# Autodesk Inventor assembly: horas_40
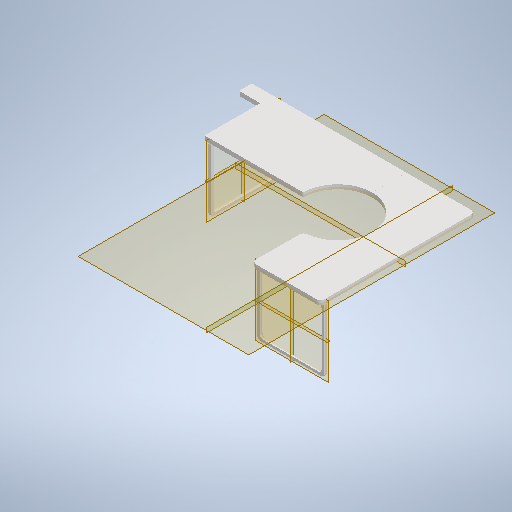
[picture p0: Inventor's stored thumbnail of the model, 512x512]
Saved by Autodesk Inventor 2025.2 (Build 292293000, 293)
## iProperties
Created: 2025-04-07
Part Number: horas_40
Document SubType Name: Assembly
Designer: kenay
Author: kenay
## Documents named in this file (4)
- C:\Users\kenay\Documents\Aula 40horas\horas_40.iam
- C:\Users\kenay\Documents\Aula 40horas\Lado Esquerdo Mesa.ipt
- C:\Users\kenay\Documents\Aula 40horas\Lado Direito Mesa.ipt
- C:\Users\kenay\Downloads\Mesa Ergonômica\Pés.ipt
## Components (4 placed, 3 different names)
1. Lado Esquerdo Mesa:1 — Alinhado:1, Alinhado:2, Alinhado:3, Coincidente:1, Coincidente:2, Alinhado:4, Coincidente:3, Alinhado:5, Alinhado:6
2. Lado Direito Mesa:1 — Coincidente:1, Coincidente:2, Alinhado:4, Alinhado:7, Coincidente:4
3. Pés:1 — Coincidente:3, Alinhado:5, Alinhado:6
4. Pés:2 — Alinhado:7, Coincidente:4
## Relationships (11: Flush 7, Mate 4)
- Alinhado:1 [Flush]: Lado Esquerdo Mesa:1
- Alinhado:2 [Flush]: Lado Esquerdo Mesa:1
- Alinhado:3 [Flush]: Lado Esquerdo Mesa:1
- Coincidente:1 [Mate]: Lado Esquerdo Mesa:1 ↔ Lado Direito Mesa:1
- Coincidente:2 [Mate]: Lado Esquerdo Mesa:1 ↔ Lado Direito Mesa:1
- Alinhado:4 [Flush]: Lado Esquerdo Mesa:1 ↔ Lado Direito Mesa:1
- Coincidente:3 [Mate]: Lado Esquerdo Mesa:1 ↔ Pés:1
- Alinhado:5 [Flush]: Lado Esquerdo Mesa:1 ↔ Pés:1
- Alinhado:6 [Flush] (-600 mm): Lado Esquerdo Mesa:1 ↔ Pés:1
- Alinhado:7 [Flush]: Lado Direito Mesa:1 ↔ Pés:2
- Coincidente:4 [Mate]: Lado Direito Mesa:1 ↔ Pés:2
